# Autodesk Inventor assembly: Rotor
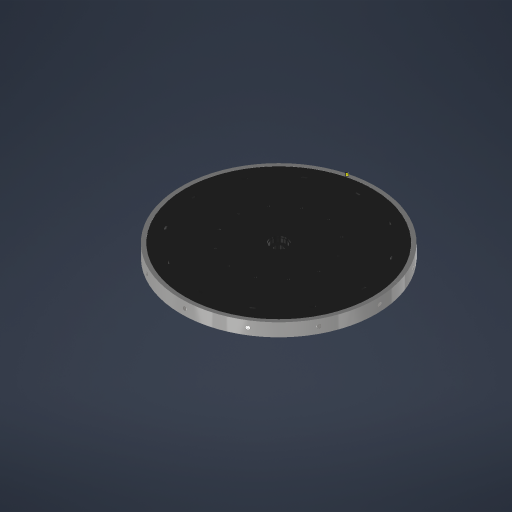
[picture p0: Inventor's stored thumbnail of the model, 512x512]
Saved by Autodesk Inventor 2023.1 (Build 271208000, 208)
## iProperties
Created: 2022-07-21
Part Number: Rotor
Document SubType Name: Assembly
Designer: ABL
Author: ABL
## Documents named in this file (15)
- C:\GitHubRepos\PHYS-12-Website\content\maker-portfolio\Axial Flux Motor\CAD\Inventor\Rotor.iam
- C:\GitHubRepos\PHYS-12-Website\content\maker-portfolio\Axial Flux Motor\CAD\Inventor\RotorBody.ipt
- C:\GitHubRepos\PHYS-12-Website\content\maker-portfolio\Axial Flux Motor\CAD\Inventor\DriveMagnet.ipt
- C:\GitHubRepos\PHYS-12-Website\content\maker-portfolio\Axial Flux Motor\CAD\Inventor\HalbachMagnet.ipt
- C:\GitHubRepos\PHYS-12-Website\content\maker-portfolio\Axial Flux Motor\CAD\Inventor\SensorMagnet.ipt
- C:\GitHubRepos\PHYS-12-Website\content\maker-portfolio\Axial Flux Motor\CAD\Inventor\SensorMagnet_Reverse.ipt
- C:\GitHubRepos\PHYS-12-Website\content\maker-portfolio\Axial Flux Motor\CAD\Inventor\DriveMagnet_Reverse.ipt
- C:\GitHubRepos\PHYS-12-Website\content\maker-portfolio\Axial Flux Motor\CAD\Inventor\HalbachMagnet_MIR1.ipt
- C:\GitHubRepos\PHYS-12-Website\content\maker-portfolio\Axial Flux Motor\CAD\Inventor\Fasteners\rotorBandBolt.ipt
- C:\GitHubRepos\PHYS-12-Website\content\maker-portfolio\Axial Flux Motor\CAD\Inventor\Fasteners\rotorBandHexNut.ipt
- C:\GitHubRepos\PHYS-12-Website\content\maker-portfolio\Axial Flux Motor\CAD\Inventor\RotorMainBody.ipt
- C:\GitHubRepos\PHYS-12-Website\content\maker-portfolio\Axial Flux Motor\CAD\Inventor\RotorBand.ipt
- C:\GitHubRepos\PHYS-12-Website\content\maker-portfolio\The Everybolt\MetricSocketBolt.ipt
- C:\GitHubRepos\PHYS-12-Website\content\maker-portfolio\The Everybolt\MetricHexNut.ipt
- C:\GitHubRepos\PHYS-12-Website\content\maker-portfolio\Axial Flux Motor\CAD\Inventor\MotorGlobalParameters.xlsx
## Components (89 placed, 11 different names)
1. RotorBody:1 — Mate:1, Mate:2, Mate:3, Mate:4, Flush:7, Mate:5, Mate:7, Mate:8, Mate:9, Angle:1, Mate:10, Mate:11, Mate:12, Mate:13, Mate:14, Mate:15, Mate:16, Flush:8, Mate:17, Mate:18, Mate:19, Mate:20, Mate:21, Mate:22, Mate:23, Mate:24
2. RotorMainBody:1 — Mate:25, Mate:26, Mate:27
3. SensorMagnet:1 — Mate:7, Mate:8
4. SensorMagnet:2
5. SensorMagnet:3
6. SensorMagnet:4
7. SensorMagnet:5
8. SensorMagnet:6
9. SensorMagnet_Reverse:1 — Mate:10, Mate:11
10. SensorMagnet_Reverse:2
11. SensorMagnet_Reverse:3
12. SensorMagnet_Reverse:4
13. SensorMagnet_Reverse:5
14. SensorMagnet_Reverse:6
15. rotorBandBolt:1 — Mate:17, Mate:18
16. rotorBandHexNut:1 — Mate:19, Mate:20, Mate:21
17. rotorBandBolt:2
18. rotorBandHexNut:2
19. rotorBandBolt:3
20. rotorBandHexNut:3
21. rotorBandBolt:4
22. rotorBandHexNut:4
23. rotorBandBolt:5
24. rotorBandHexNut:5
25. rotorBandBolt:6
26. rotorBandHexNut:6
27. rotorBandBolt:7
28. rotorBandHexNut:7
29. rotorBandBolt:8
30. rotorBandHexNut:8
31. rotorBandBolt:9
32. rotorBandHexNut:9
33. rotorBandBolt:10
34. rotorBandHexNut:10
35. rotorBandBolt:11
36. rotorBandHexNut:11
37. rotorBandBolt:12
38. rotorBandHexNut:12
39. RotorBand:1 — Mate:28, Mate:29, Mate:30
40. RotorBand:2
41. RotorBand:3
42. DriveMagnet:1 — Mate:1, Mate:2, Mate:3
43. DriveMagnet:2
44. HalbachMagnet:1 — Mate:4, Flush:7, Mate:5
45. HalbachMagnet:2
46. DriveMagnet:3
47. DriveMagnet:4
48. HalbachMagnet:3
49. HalbachMagnet:4
50. DriveMagnet:5
51. DriveMagnet:6
52. HalbachMagnet:5
53. HalbachMagnet:6
54. DriveMagnet:7
55. DriveMagnet:8
56. HalbachMagnet:7
57. HalbachMagnet:8
58. DriveMagnet:9
59. DriveMagnet:10
60. HalbachMagnet:9
61. HalbachMagnet:10
62. DriveMagnet:11
63. DriveMagnet:12
64. HalbachMagnet:11
65. HalbachMagnet:12
66. DriveMagnet_Reverse:1 — Mate:12, Mate:13, Mate:14
67. DriveMagnet_Reverse:2
68. HalbachMagnet_MIR1:1
69. HalbachMagnet_MIR1:2 — Mate:15, Mate:16, Flush:8
70. DriveMagnet_Reverse:3
71. DriveMagnet_Reverse:4
72. HalbachMagnet_MIR1:3
73. HalbachMagnet_MIR1:4
74. DriveMagnet_Reverse:5
75. DriveMagnet_Reverse:6
76. HalbachMagnet_MIR1:5
77. HalbachMagnet_MIR1:6
78. DriveMagnet_Reverse:7
79. DriveMagnet_Reverse:8
80. HalbachMagnet_MIR1:7
81. HalbachMagnet_MIR1:8
82. DriveMagnet_Reverse:9 — Symmetry:1
83. DriveMagnet_Reverse:10 — Symmetry:1
84. HalbachMagnet_MIR1:9
85. HalbachMagnet_MIR1:10
86. DriveMagnet_Reverse:11
87. DriveMagnet_Reverse:12
88. HalbachMagnet_MIR1:11
89. HalbachMagnet_MIR1:12
## Component patterns: NorthMagnets (6 elements), SouthMagnets (6 elements), (12 elements, first: rotorBandBolt:1 + rotorBandHexNut:1), (3 elements, first: RotorBand:1), DriveMagnetStack (2 elements), HalbachMagnetStack (2 elements), DriveMagnetStack:2 (2 elements), HalbachMagnetStack:2 (2 elements), DriveMagnetStack:3 (2 elements), HalbachMagnetStack:3 (2 elements), DriveMagnetStack:4 (2 elements), HalbachMagnetStack:4 (2 elements), DriveMagnetStack:5 (2 elements), HalbachMagnetStack:5 (2 elements), DriveMagnetStack:6 (2 elements), HalbachMagnetStack:6 (2 elements), DriveMagnetStack_Reverse (2 elements), HalbachMagnetStack_Reverse (2 elements), (2 elements, first: DriveMagnet_Reverse:3), (2 elements, first: HalbachMagnet_MIR1:3), (2 elements, first: DriveMagnet_Reverse:5), (2 elements, first: HalbachMagnet_MIR1:5), (2 elements, first: DriveMagnet_Reverse:7), (2 elements, first: HalbachMagnet_MIR1:7), (2 elements, first: DriveMagnet_Reverse:9), (2 elements, first: HalbachMagnet_MIR1:9), (2 elements, first: DriveMagnet_Reverse:11), (2 elements, first: HalbachMagnet_MIR1:11)
## Relationships (33: Mate 29, Flush 2, Angle 1, Symmetry 1)
- Mate:1: RotorBody:1 ↔ DriveMagnet:1
- Mate:2 (0.1 mm): RotorBody:1 ↔ DriveMagnet:1
- Mate:3 (0.1 mm): RotorBody:1 ↔ DriveMagnet:1
- Mate:4 (0.1 mm): RotorBody:1 ↔ HalbachMagnet:1
- Flush:7 (0.1 mm): RotorBody:1 ↔ HalbachMagnet:1
- Mate:5: RotorBody:1 ↔ HalbachMagnet:1
- Mate:7: RotorBody:1 ↔ SensorMagnet:1
- Mate:8: RotorBody:1 ↔ SensorMagnet:1
- Mate:9: RotorBody:1
- Angle:1 (90 deg): RotorBody:1
- Mate:10: RotorBody:1 ↔ SensorMagnet_Reverse:1
- Mate:11: RotorBody:1 ↔ SensorMagnet_Reverse:1
- Mate:12: RotorBody:1 ↔ DriveMagnet_Reverse:1
- Mate:13 (0.1 mm): RotorBody:1 ↔ DriveMagnet_Reverse:1
- Mate:14 (0.1 mm): RotorBody:1 ↔ DriveMagnet_Reverse:1
- Mate:15 (0.1 mm): RotorBody:1 ↔ HalbachMagnet_MIR1:2
- Mate:16: RotorBody:1 ↔ HalbachMagnet_MIR1:2
- Flush:8 (0.1 mm): RotorBody:1 ↔ HalbachMagnet_MIR1:2
- Mate:17: RotorBody:1 ↔ rotorBandBolt:1
- Mate:18: RotorBody:1 ↔ rotorBandBolt:1
- Mate:19: RotorBody:1 ↔ rotorBandHexNut:1
- Mate:20 (0.2 mm): RotorBody:1 ↔ rotorBandHexNut:1
- Mate:21: RotorBody:1 ↔ rotorBandHexNut:1
- Mate:22: RotorBody:1
- Mate:23: RotorBody:1
- Mate:24: RotorBody:1
- Mate:25: RotorMainBody:1
- Mate:26: RotorMainBody:1
- Mate:27: RotorMainBody:1
- Mate:28: RotorBand:1
- Mate:29: RotorBand:1
- Mate:30: RotorBand:1
- Symmetry:1: DriveMagnet_Reverse:9 ↔ DriveMagnet_Reverse:10
## Named parameters: gap = 0.1 mm, airgap = 0.4 mm, driveMagnet_length = 60 mm, driveMagnet_width = 10 mm, driveMagnet_height = 5 mm, halbachMagnet_length = 60 mm, halbachMagnet_width = 10 mm, halbachMagnet_height = 3 mm, sensorMagnet_diameter = 5 mm, sensorMagnet_height = 2.66667 mm, numMagnetSets = 12, numElectromagnets = 9, wallgap = 2 mm, halbachMagnet_numStacked = 2, driveMagnet_centerSpacingRadius = 38.96113 mm, motorRadius = 103.16113 mm, rotorThickness = 14.1 mm, driveMagnet_numStacked = 2, shaftDiameter = 8 mm, flangeBearing_outerDiameter = 16 mm, flangeBearing_innerDiameter = 8 mm, flangeBearing_height = 5 mm, flangeBearing_flangeHeight = 1 mm, flangeBearing_flangeDiameter = 18 mm, magnetTrapNut_height = 1.2 mm, magnetTrapNut_sideToSide = 4 mm, magnetTrapBolt_headHeight = 2 mm, magnetTrapBolt_headDiameter = 3.98 mm, magnetTrapBolt_diameter = 2 mm, statorThickness = 16 mm, rotor_mountingLipHeight = 8 mm, magnetTrapBolt_shaftLength = 20 mm, magnetTrapHexNut_sideToSide = 4 mm, magnetTrapSquareNut_sideLength = 4 mm, magnetTrapSquareNut_height = 1.2 mm, magnetTrapHexNut_height = 1.2 mm, magnetTrap_wingDegrees = 4.443207 deg, magnetTrap_wingOuterDegrees = 11.764706 deg, rotorRadius = 101.16113 mm, rotorBandSquareNut_sideLength = 4 mm, rotorBandHexNut_height = 1.2 mm, rotorBandBolt_shaftLength = 20 mm, rotorBandHexNut_sideToSide = 4 mm, rotorBandSquareNut_height = 1.2 mm, rotorBandBolt_headHeight = 2 mm, rotorBandBolt_headDiameter = 3.98 mm, rotorBandBolt_diameter = 2 mm, rotorBandThickness = 4.1 mm, shaftLength = 200 mm, flangeCoupling_collarOuterDiameter = 16 mm, flangeCoupling_flangeHoleEdgeToEdge = 2.05 mm, flangeCoupling_innerDiameter = 8 mm, flangeCoupling_flangeHoleDiameter = 3.9 mm, flangeCoupling_flangeHeight = 3.1 mm, flangeCoupling_collarHeight = 10 mm, flangeCoupling_flangeDiameter = 32 mm, flangeCoupling_height = 13.1 mm, flangeCoupling_mountHoleDiameter = 3.9 mm, flangeCoupling_mountHoleEdgeToEdge = 2.05 mm, statorRadius = 99.16113 mm, coilThickness = 12 mm, statorMountBolt_diameter = 4 mm, statorMountBolt_headDiameter = 7 mm, statorMountBolt_headHeight = 4 mm, statorMountBolt_shaftLength = 17.1 mm, statorMountHexNut_height = 4 mm, statorMountHexNut_sideToSide = 8 mm, sensorMagnet_ringRadius = 23.48057 mm, coil_percentCoverage = 0.6, statorSpokeDegrees = 4 deg, coil_bulge = 3 mm, coil_cornerRadius = 10 mm, coil_width = 10 mm, statorCoilBolt_shaftLength = 19.3 mm, statorCoilHexNut_height = 1.2 mm, statorCoilBolt_headHeight = 2 mm, statorCoilBolt_diameter = 2 mm, statorCoilBolt_headDiameter = 3.98 mm, statorCoilHexNut_sideToSide = 4 mm, magnetWire_gauge = 20, magnetWire_outerDiameter = 0.8128 mm, printingLayerHeight = 0.2 mm, circuitBoard_height = 1.6 mm, hallEffectSensor_width = 1.6 mm, hallEffectSensor_length = 3 mm, hallEffectSensor_height = 1.1 mm, hallEffectSensor_pinLength = 0.6 mm, circuitboardMountHexNut_height = 1.2 mm, circuitboardMountHexNut_sideToSide = 4 mm, circuitboardMountBolt_headHeight = 2 mm, circuitboardMountBolt_shaftLength = 12 mm, circuitboardMountBolt_diameter = 2 mm, circuitboardMountBolt_headDiameter = 3.98 mm, statorShellBolt_headDiameter = 5.68 mm, statorShellHexNut_height = 2.3 mm, statorShellBolt_shaftLength = 12.6 mm, statorShellBolt_headHeight = 3 mm, statorShellHexNut_sideToSide = 5.3 mm, statorShellBolt_diameter = 3 mm, statorShellBolt_countersinkDepth = 3.4 mm, flangeCoupling_mountHoleCenterToCouplingCenter = 12 mm
